# Autodesk Inventor assembly: axis assembly
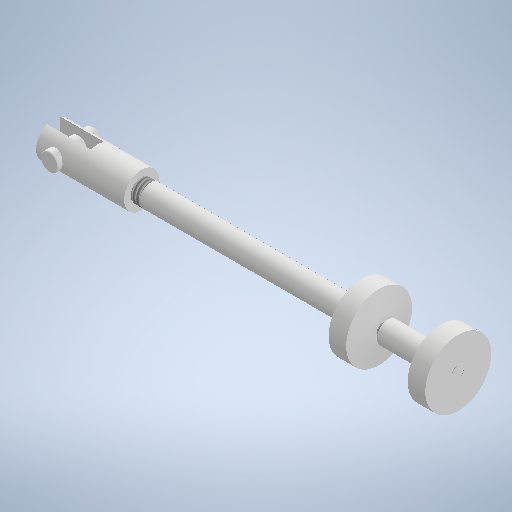
[picture p0: Inventor's stored thumbnail of the model, 512x512]
Saved by Autodesk Inventor 2025.1 (Build 291241000, 241)
## iProperties
Created: 2024-09-18
Part Number: axis assembly
Document SubType Name: Assembly
Designer: ffogue
Author: ffogue
## Documents named in this file (6)
- C:\Users\ffogue\Documents\Inventor\Cylinder Radial Steam Engine\axis assembly.iam
- C:\Users\ffogue\Documents\Inventor\Cylinder Radial Steam Engine\19.ipt
- C:\Users\ffogue\Documents\Inventor\Cylinder Radial Steam Engine\17.ipt
- C:\Users\ffogue\Documents\Inventor\Cylinder Radial Steam Engine\20.ipt
- C:\Users\ffogue\Documents\Inventor\Cylinder Radial Steam Engine\21.ipt
- C:\Users\ffogue\Documents\Inventor\Cylinder Radial Steam Engine\22.ipt
## Components (6 placed, 5 different names)
1. 19:1 — Mate:4, Insert:4, Angle:1, Mate:5, Flush:1, Mate:6, Insert:5, Mate:7
2. 17:1 — Mate:4, Insert:4, Angle:1, Mate:8, Rotational:1
3. 20:1 — Mate:5, Flush:1
4. 20:2 — Mate:6, Insert:5, Insert:6
5. 21:1 — Mate:7, Insert:6
6. 22:1 — Mate:8, Rotational:1
## Relationships (11: Mate 5, Insert 3, Angle 1, Flush 1, RevoluteJoint 1)
- Mate:4: 19:1 ↔ 17:1
- Insert:4 (-8 mm): 19:1 ↔ 17:1
- Angle:1 (0 deg): 19:1 ↔ 17:1
- Mate:5: 19:1 ↔ 20:1
- Flush:1: 19:1 ↔ 20:1
- Mate:6: 19:1 ↔ 20:2
- Insert:5: 19:1 ↔ 20:2
- Mate:7: 19:1 ↔ 21:1
- Insert:6 (1 mm): 20:2 ↔ 21:1
- Mate:8: 17:1 ↔ 22:1
- Rotational:1 [RevoluteJoint] (-8.5 mm): 17:1 ↔ 22:1
